# Autodesk Inventor assembly: moteur
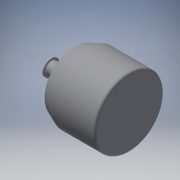
[picture p0: Inventor's stored thumbnail of the model, 180x180]
Saved by Autodesk Inventor 2018.1 (Build 221171000, 171)
## iProperties
Created: 2022-06-30
Part Number: moteur
Document SubType Name: Assembly
Designer: mouta
Author: mouta
## Documents named in this file (3)
- C:\Users\Bureau\Mon Drive\Manu\USINAGE\MoteurVelo\Moteur\moteur.iam
- C:\Users\Bureau\Mon Drive\Manu\USINAGE\MoteurVelo\Moteur\moteur.ipt
- C:\Users\Bureau\Mon Drive\Manu\USINAGE\MoteurVelo\Moteur\pignon 12 dents.ipt
## Components (2 placed, 2 different names)
1. moteur:1 — Mate:1, Mate:2
2. pignon 12 dents:1 — Mate:1, Mate:2
## Relationships (2: Mate 2)
- Mate:1: moteur:1 ↔ pignon 12 dents:1
- Mate:2: moteur:1 ↔ pignon 12 dents:1
